# Autodesk Inventor assembly: 000.005 -  Манипулятор
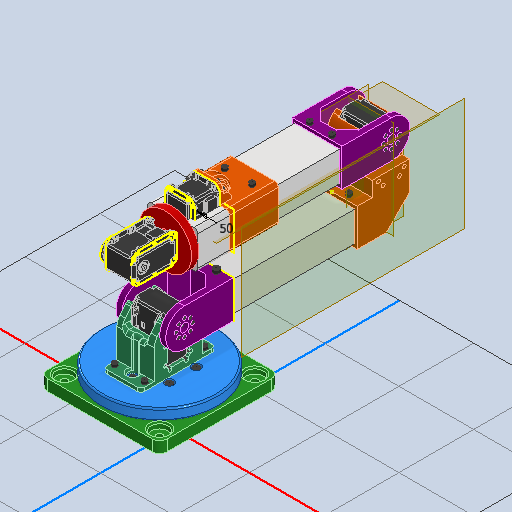
[picture p0: Inventor's stored thumbnail of the model, 512x512]
Saved by Autodesk Inventor 2022 (Build 260153000, 153)
## iProperties
Created: 2022-11-17
Part Number: 000.005 -  Манипулятор
Document SubType Name: Assembly
Designer: Petrov Ivan
Mass: 2206.34 g
Surface Area: 5807.56 cm^2
Volume: 1972.51 cm^3
Density: 1.11854 g/cm^3
Author: Petrov Ivan
## Documents named in this file (8)
- D:\IVAN\Ivan_desktop\Kvantorium\Projects\YouBotRobot\design\000.005 -  Манипулятор.iam
- D:\IVAN\Ivan_desktop\Kvantorium\Projects\YouBotRobot\design\000.005.001 - Поворотный стол.iam
- D:\IVAN\Ivan_desktop\Kvantorium\Projects\YouBotRobot\design\000.005.002 - Плечо СБ.iam
- D:\IVAN\Ivan_desktop\Kvantorium\Projects\YouBotRobot\design\000.005.003 - Локоть СБ.iam
- D:\IVAN\Ivan_desktop\Kvantorium\Projects\YouBotRobot\design\Content Center Files\R2022\ru-RU\ISO 4762(1)\DIN EN ISO 4762 - M4 x 16.ipt
- D:\IVAN\Ivan_desktop\Kvantorium\Projects\YouBotRobot\design\000.005.004 - Поворот сгиба кисти СБ.iam
- D:\IVAN\Ivan_desktop\Kvantorium\Projects\YouBotRobot\design\Content Center Files\R2022\ru-RU\BS EN 24035\ISO 4035 - M2.5BS EN.ipt
- D:\IVAN\Ivan_desktop\Kvantorium\Projects\YouBotRobot\design\Content Center Files\R2022\ru-RU\ISO 4762(1)\DIN EN ISO 4762 - M2.5 x 10.ipt
## Components (20 placed, 7 different names)
1. 000.005.001 - Поворотный стол СБ:1 [sub-assembly] — Совмещение:1, Совмещение:2, Совмещение:3, Угол:1, Угол:2
2. 000.005.002 - Плечо СБ:1 [sub-assembly] — Совмещение:1, Совмещение:2, Совмещение:3, Вставка:1, Вставка:2, Вставка:3, Вставка:4, Угол:1, Совмещение:4, Совмещение:5, Совмещение:6, Угол:2, Угол:3
3. 000.005.003 - Локоть СБ:1 [sub-assembly] — Совмещение:4, Совмещение:5, Совмещение:6, Угол:3, Угол:4, Угол:5, Совмещение:7, Совмещение:8, Совмещение:9
4. DIN EN ISO 4762 M4 x 16:1 — Вставка:1
5. DIN EN ISO 4762 M4 x 16:2 — Вставка:2
6. DIN EN ISO 4762 M4 x 16:3 — Вставка:3
7. DIN EN ISO 4762 M4 x 16:4 — Вставка:4
8. 000.005.004 - Поворот сгиба кисти СБ:1 [sub-assembly] — Совмещение:7, Совмещение:8, Совмещение:9, Вставка:5, Вставка:6, Вставка:7, Вставка:8, Вставка:9, Вставка:10, Вставка:11, Вставка:12, Вставка:13, Вставка:14, Вставка:15, Вставка:16
9. BS EN 24035 - метрическая M2,5:1 — Вставка:5
10. BS EN 24035 - метрическая M2,5:2 — Вставка:6
11. BS EN 24035 - метрическая M2,5:3 — Вставка:7
12. BS EN 24035 - метрическая M2,5:4 — Вставка:8
13. BS EN 24035 - метрическая M2,5:5 — Вставка:9
14. BS EN 24035 - метрическая M2,5:6 — Вставка:10
15. BS EN 24035 - метрическая M2,5:7 — Вставка:11
16. BS EN 24035 - метрическая M2,5:8 — Вставка:12
17. DIN EN ISO 4762 M2,5 x 10:1 — Вставка:13
18. DIN EN ISO 4762 M2,5 x 10:2 — Вставка:14
19. DIN EN ISO 4762 M2,5 x 10:3 — Вставка:15
20. DIN EN ISO 4762 M2,5 x 10:4 — Вставка:16
## Relationships (30: Insert 16, Mate 9, Angle 5)
- Совмещение:1 [Mate]: 000.005.001 - Поворотный стол СБ:1 ↔ 000.005.002 - Плечо СБ:1
- Совмещение:2 [Mate]: 000.005.001 - Поворотный стол СБ:1 ↔ 000.005.002 - Плечо СБ:1
- Совмещение:3 [Mate]: 000.005.001 - Поворотный стол СБ:1 ↔ 000.005.002 - Плечо СБ:1
- Вставка:1 [Insert]: 000.005.002 - Плечо СБ:1 ↔ DIN EN ISO 4762 M4 x 16:1
- Вставка:2 [Insert]: 000.005.002 - Плечо СБ:1 ↔ DIN EN ISO 4762 M4 x 16:2
- Вставка:3 [Insert]: 000.005.002 - Плечо СБ:1 ↔ DIN EN ISO 4762 M4 x 16:3
- Вставка:4 [Insert]: 000.005.002 - Плечо СБ:1 ↔ DIN EN ISO 4762 M4 x 16:4
- Угол:1 [Angle] (180 deg): 000.005.001 - Поворотный стол СБ:1 ↔ 000.005.002 - Плечо СБ:1
- Совмещение:4 [Mate]: 000.005.002 - Плечо СБ:1 ↔ 000.005.003 - Локоть СБ:1
- Совмещение:5 [Mate] (0.25 mm): 000.005.002 - Плечо СБ:1 ↔ 000.005.003 - Локоть СБ:1
- Совмещение:6 [Mate] (0.25 mm): 000.005.002 - Плечо СБ:1 ↔ 000.005.003 - Локоть СБ:1
- Угол:2 [Angle] (0 deg): 000.005.001 - Поворотный стол СБ:1 ↔ 000.005.002 - Плечо СБ:1
- Угол:3 [Angle] (0 deg): 000.005.002 - Плечо СБ:1 ↔ 000.005.003 - Локоть СБ:1
- Угол:4 [Angle] (0 deg): 000.005.003 - Локоть СБ:1
- Угол:5 [Angle] (0 deg): 000.005.003 - Локоть СБ:1
- Совмещение:7 [Mate]: 000.005.003 - Локоть СБ:1 ↔ 000.005.004 - Поворот сгиба кисти СБ:1
- Совмещение:8 [Mate]: 000.005.003 - Локоть СБ:1 ↔ 000.005.004 - Поворот сгиба кисти СБ:1
- Совмещение:9 [Mate]: 000.005.003 - Локоть СБ:1 ↔ 000.005.004 - Поворот сгиба кисти СБ:1
- Вставка:5 [Insert]: 000.005.004 - Поворот сгиба кисти СБ:1 ↔ BS EN 24035 - метрическая M2,5:1
- Вставка:6 [Insert]: 000.005.004 - Поворот сгиба кисти СБ:1 ↔ BS EN 24035 - метрическая M2,5:2
- Вставка:7 [Insert]: 000.005.004 - Поворот сгиба кисти СБ:1 ↔ BS EN 24035 - метрическая M2,5:3
- Вставка:8 [Insert]: 000.005.004 - Поворот сгиба кисти СБ:1 ↔ BS EN 24035 - метрическая M2,5:4
- Вставка:9 [Insert]: 000.005.004 - Поворот сгиба кисти СБ:1 ↔ BS EN 24035 - метрическая M2,5:5
- Вставка:10 [Insert]: 000.005.004 - Поворот сгиба кисти СБ:1 ↔ BS EN 24035 - метрическая M2,5:6
- Вставка:11 [Insert]: 000.005.004 - Поворот сгиба кисти СБ:1 ↔ BS EN 24035 - метрическая M2,5:7
- Вставка:12 [Insert]: 000.005.004 - Поворот сгиба кисти СБ:1 ↔ BS EN 24035 - метрическая M2,5:8
- Вставка:13 [Insert]: 000.005.004 - Поворот сгиба кисти СБ:1 ↔ DIN EN ISO 4762 M2,5 x 10:1
- Вставка:14 [Insert]: 000.005.004 - Поворот сгиба кисти СБ:1 ↔ DIN EN ISO 4762 M2,5 x 10:2
- Вставка:15 [Insert]: 000.005.004 - Поворот сгиба кисти СБ:1 ↔ DIN EN ISO 4762 M2,5 x 10:3
- Вставка:16 [Insert]: 000.005.004 - Поворот сгиба кисти СБ:1 ↔ DIN EN ISO 4762 M2,5 x 10:4
